# Autodesk Inventor assembly: base mg996r 3mm frame bottom
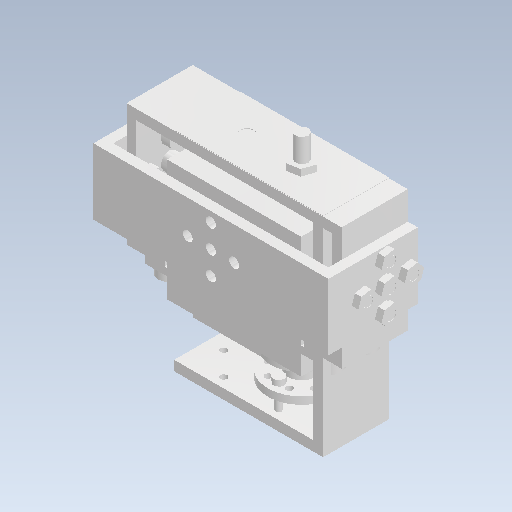
[picture p0: Inventor's stored thumbnail of the model, 512x512]
Saved by Autodesk Inventor 2021.4 (Build 254397000, 397)
## iProperties
Created: 2022-07-09
Part Number: base mg996r 3mm frame bottom
Document SubType Name: Assembly
Designer: isamu
Author: isamu
## Documents named in this file (5)
- D:\personal_projects\robot\inventor\2021\base mg996r 3mm frame bottom.iam
- D:\personal_projects\robot\inventor\2021\base mg996r 3mm frame with axis.iam
- D:\personal_projects\robot\exports\frames\servo frame part 3.ipt
- D:\personal_projects\robot\exports\screws\m3x8.ipt
- D:\personal_projects\robot\exports\screws\m3 nuts.ipt
## Components (22 placed, 4 different names)
1. base mg996r 3mm frame with axis:1 [sub-assembly] — Mate:1, Mate:2, Mate:3, Insert:1, Insert:2, Insert:3, Insert:4, Insert:5, Insert:6, Insert:7, Insert:8, Insert:9, Insert:10
2. servo frame part 3:1 — Mate:1, Mate:2, Mate:3, Insert:11, Insert:12, Insert:13, Insert:14, Insert:15, Insert:16, Insert:17, Insert:18, Insert:19, Insert:20
3. m3x8:1 — Insert:4
4. m3x8:2 — Insert:7
5. m3x8:3 — Insert:6
6. m3x8:4 — Insert:1
7. m3x8:5 — Insert:5
8. m3x8:6 — Insert:2
9. m3x8:7 — Insert:8
10. m3x8:8 — Insert:9
11. m3x8:9 — Insert:10
12. m3x8:10 — Insert:3
13. m3 nuts:1 — Insert:11
14. m3 nuts:2 — Insert:14
15. m3 nuts:3 — Insert:12
16. m3 nuts:4 — Insert:16
17. m3 nuts:5 — Insert:13
18. m3 nuts:6 — Insert:15
19. m3 nuts:7 — Insert:17
20. m3 nuts:8 — Insert:18
21. m3 nuts:9 — Insert:20
22. m3 nuts:10 — Insert:19
## Relationships (23: Insert 20, Mate 3)
- Mate:1: base mg996r 3mm frame with axis:1 ↔ servo frame part 3:1
- Mate:2: base mg996r 3mm frame with axis:1 ↔ servo frame part 3:1
- Mate:3: base mg996r 3mm frame with axis:1 ↔ servo frame part 3:1
- Insert:1: base mg996r 3mm frame with axis:1 ↔ m3x8:4
- Insert:2: base mg996r 3mm frame with axis:1 ↔ m3x8:6
- Insert:3: base mg996r 3mm frame with axis:1 ↔ m3x8:10
- Insert:4: base mg996r 3mm frame with axis:1 ↔ m3x8:1
- Insert:5: base mg996r 3mm frame with axis:1 ↔ m3x8:5
- Insert:6: base mg996r 3mm frame with axis:1 ↔ m3x8:3
- Insert:7: base mg996r 3mm frame with axis:1 ↔ m3x8:2
- Insert:8: base mg996r 3mm frame with axis:1 ↔ m3x8:7
- Insert:9: base mg996r 3mm frame with axis:1 ↔ m3x8:8
- Insert:10: base mg996r 3mm frame with axis:1 ↔ m3x8:9
- Insert:11: servo frame part 3:1 ↔ m3 nuts:1
- Insert:12: servo frame part 3:1 ↔ m3 nuts:3
- Insert:13: servo frame part 3:1 ↔ m3 nuts:5
- Insert:14: servo frame part 3:1 ↔ m3 nuts:2
- Insert:15: servo frame part 3:1 ↔ m3 nuts:6
- Insert:16: servo frame part 3:1 ↔ m3 nuts:4
- Insert:17: servo frame part 3:1 ↔ m3 nuts:7
- Insert:18: servo frame part 3:1 ↔ m3 nuts:8
- Insert:19: servo frame part 3:1 ↔ m3 nuts:10
- Insert:20: servo frame part 3:1 ↔ m3 nuts:9
